# Autodesk Inventor assembly: Collector Arms v2.0_MIR_MIR_MIR2_MIR
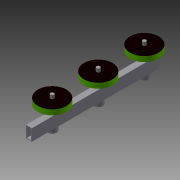
[picture p0: Inventor's stored thumbnail of the model, 180x180]
Saved by Autodesk Inventor 2015 (Build 190159000, 159)
## iProperties
Created: 2015-01-20
Part Number: Collector Arms v2.0_MIR_MIR_MIR2_MIR
Document SubType Name: Assembly
Designer: szymsea16
Author: chapale16
## Documents named in this file (4)
- \\lhssvr02\Homedirs\Robotics Club\CAD Model 2015\CDR prep\Tote Collector Arms\Collector Arms v2.0_MIR_MIR_MIR2_MIR.iam
- \\lhssvr02\Homedirs\Robotics Club\CAD Model 2015\CDR prep\Tote Collector Arms\23.5 in 2 x 1 boxBeam_MIR_MIR_MIR2_MIR.ipt
- \\lhssvr02\Homedirs\Robotics Club\CAD Model 2015\CDR prep\Tote Collector Arms\collector arm wheel_MIR2_MIR_MIR2_MIR.ipt
- \\lhssvr02\Homedirs\Robotics Club\CAD Model 2015\CDR prep\Tote Collector Arms\P60 Gear Box_MIR2_MIR_MIR2_MIR.ipt
## Components (7 placed, 3 different names)
1. 23.5 in 2 x 1 boxBeam_MIR_MIR_MIR2_MIR:1 — Mate:4, Mate:3, Mate:2, Mate:7, Mate:6, Mate:5, Mate:10, Mate:9, Mate:8
2. collector arm wheel_MIR2_MIR_MIR2_MIR:1 — Mate:1, Flush:1
3. P60 Gear Box_MIR2_MIR_MIR2_MIR:1 — Mate:4, Mate:3, Mate:2, Mate:1
4. P60 Gear Box_MIR2_MIR_MIR2_MIR:2 — Mate:7, Mate:6, Mate:5, Mate:11
5. P60 Gear Box_MIR2_MIR_MIR2_MIR:3 — Mate:10, Mate:9, Mate:8, Mate:12
6. collector arm wheel_MIR2_MIR_MIR2_MIR:2 — Flush:1, Mate:11, Flush:2
7. collector arm wheel_MIR2_MIR_MIR2_MIR:3 — Flush:2, Mate:12
## Relationships (14: Mate 12, Flush 2)
- Mate:4: 23.5 in 2 x 1 boxBeam_MIR_MIR_MIR2_MIR:1 ↔ P60 Gear Box_MIR2_MIR_MIR2_MIR:1
- Mate:3: 23.5 in 2 x 1 boxBeam_MIR_MIR_MIR2_MIR:1 ↔ P60 Gear Box_MIR2_MIR_MIR2_MIR:1
- Mate:2: 23.5 in 2 x 1 boxBeam_MIR_MIR_MIR2_MIR:1 ↔ P60 Gear Box_MIR2_MIR_MIR2_MIR:1
- Mate:1: collector arm wheel_MIR2_MIR_MIR2_MIR:1 ↔ P60 Gear Box_MIR2_MIR_MIR2_MIR:1
- Mate:7: 23.5 in 2 x 1 boxBeam_MIR_MIR_MIR2_MIR:1 ↔ P60 Gear Box_MIR2_MIR_MIR2_MIR:2
- Mate:6: 23.5 in 2 x 1 boxBeam_MIR_MIR_MIR2_MIR:1 ↔ P60 Gear Box_MIR2_MIR_MIR2_MIR:2
- Mate:5: 23.5 in 2 x 1 boxBeam_MIR_MIR_MIR2_MIR:1 ↔ P60 Gear Box_MIR2_MIR_MIR2_MIR:2
- Mate:10: 23.5 in 2 x 1 boxBeam_MIR_MIR_MIR2_MIR:1 ↔ P60 Gear Box_MIR2_MIR_MIR2_MIR:3
- Mate:9: 23.5 in 2 x 1 boxBeam_MIR_MIR_MIR2_MIR:1 ↔ P60 Gear Box_MIR2_MIR_MIR2_MIR:3
- Mate:8: 23.5 in 2 x 1 boxBeam_MIR_MIR_MIR2_MIR:1 ↔ P60 Gear Box_MIR2_MIR_MIR2_MIR:3
- Flush:1: collector arm wheel_MIR2_MIR_MIR2_MIR:1 ↔ collector arm wheel_MIR2_MIR_MIR2_MIR:2
- Mate:11: P60 Gear Box_MIR2_MIR_MIR2_MIR:2 ↔ collector arm wheel_MIR2_MIR_MIR2_MIR:2
- Flush:2: collector arm wheel_MIR2_MIR_MIR2_MIR:2 ↔ collector arm wheel_MIR2_MIR_MIR2_MIR:3
- Mate:12: P60 Gear Box_MIR2_MIR_MIR2_MIR:3 ↔ collector arm wheel_MIR2_MIR_MIR2_MIR:3
